# Autodesk Inventor assembly: DC15_A01_DUMMY_ASSY_IDLE_ASM
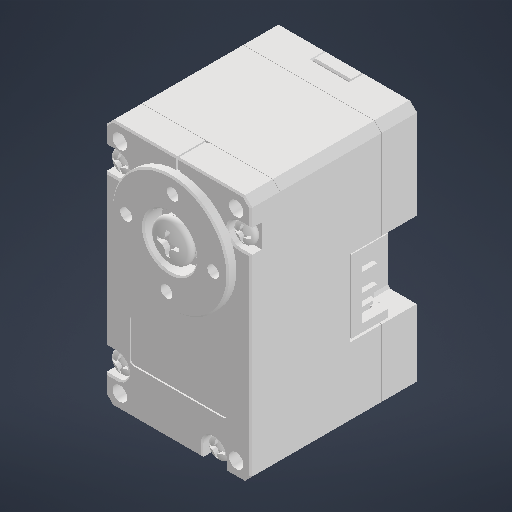
[picture p0: Inventor's stored thumbnail of the model, 512x512]
Saved by Autodesk Inventor 2026 (Build 300175000, 175)
## iProperties
Created: 2020-07-27
Part Number: DC15_A01_DUMMY_ASSY_IDLE_ASM
Document SubType Name: Assembly
Designer: Yueda
Sending System: CREO PARAMETRIC BY PTC INC, 2019224
Preprocessor: CREO PARAMETRIC BY PTC INC, 2019224
Title: DC15_A01_DUMMY_ASSY_IDLE_ASM
Author: yunever
Revision Number: 9LAST_VERSION
## Documents named in this file (9)
- C:\Users\Elizabeth\FrontierLab\firstMockup\DYNAMIXEL\DYNAMIXEL_XL330XL,XC-330.iam
- C:\Users\Elizabeth\FrontierLab\firstMockup\DYNAMIXEL\DYNAMIXEL_XL330DC15_A01_CASE_M_DUMMY.ipt
- C:\Users\Elizabeth\FrontierLab\firstMockup\DYNAMIXEL\DYNAMIXEL_XL330DC15_A01_CASE_F_DUMMY.ipt
- C:\Users\Elizabeth\FrontierLab\firstMockup\DYNAMIXEL\DYNAMIXEL_XL330DC15_A01_CASE_B_DUMMY.ipt
- C:\Users\Elizabeth\FrontierLab\firstMockup\DYNAMIXEL\DYNAMIXEL_XL330DC15_A01_LED_CAP2_DUMMY.ipt
- C:\Users\Elizabeth\FrontierLab\firstMockup\DYNAMIXEL\DYNAMIXEL_XL330PHS_1_7X20_5_DC10.ipt
- C:\Users\Elizabeth\FrontierLab\firstMockup\DYNAMIXEL\DYNAMIXEL_XL330BTS2_M2_6X8.ipt
- C:\Users\Elizabeth\FrontierLab\firstMockup\DYNAMIXEL\DYNAMIXEL_XL330B3B-EH.ipt
- C:\Users\Elizabeth\FrontierLab\firstMockup\DYNAMIXEL\DYNAMIXEL_XL330DC15_A01_HORN_IDLE2_DUMMY.ipt
## Components (12 placed, 12 different names)
1. 0 — Mate:1, Mate:3, Mate:4
2. 1 — Mate:2
3. 2
4. 4
5. 5
6. 6
7. 7
8. 8
9. 9 — Mate:3, Mate:4
10. 13
11. 14
12. DYNAMIXEL_XL330DC15_A01_HORN_IDLE2_DUMMY:1 — Mate:1, Mate:2
## Relationships (4: Mate 4)
- Mate:1: 0 ↔ DYNAMIXEL_XL330DC15_A01_HORN_IDLE2_DUMMY:1
- Mate:2: 1 ↔ DYNAMIXEL_XL330DC15_A01_HORN_IDLE2_DUMMY:1
- Mate:3: 0 ↔ 9
- Mate:4: 0 ↔ 9
